# Autodesk Inventor assembly: outer_MIR
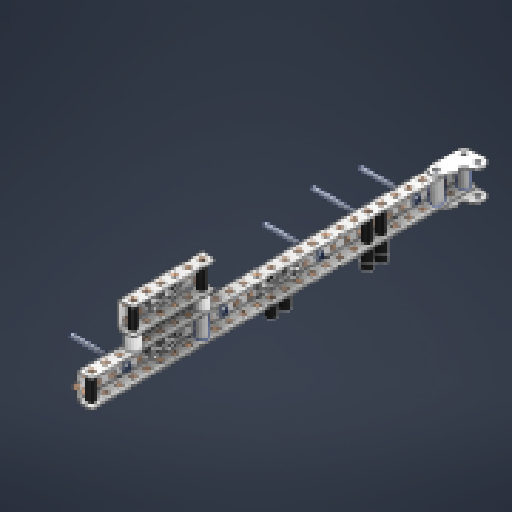
[picture p0: Inventor's stored thumbnail of the model, 512x512]
Saved by Autodesk Inventor 2024 (Build 280153000, 153)
## iProperties
Created: 2023-10-18
Part Number: outer_MIR
Document SubType Name: Assembly
Designer: Averey Ku
Author: avere
## Documents named in this file (16)
- D:\vex_robotics\hardware\cad\goated_v0.1\chassis\mirrored_parts\outer_MIR.iam
- D:\vex_robotics\hardware\cad\goated_v0.1\chassis\mirrored_parts\Alu C 1x2x1x28_MIR.ipt
- D:\vex_robotics\hardware\cad\goated_v0.1\chassis\mirrored_parts\Alu C 1x2x1x6_MIR.ipt
- D:\vex_robotics\hardware\cad\goated_v0.1\chassis\mirrored_parts\lightweight_offset_bearing_MIR.iam
- D:\vex_robotics\hardware\cad\goated_v0.1\chassis\mirrored_parts\.375 OD Aluminum Spacer 0.875_MIR.ipt
- D:\vex_robotics\hardware\cad\VEX-CAD-Inventor-1.41\Structure\Standoff\Standoff .875.ipt
- D:\vex_robotics\hardware\cad\VEX-CAD-Inventor-1.41\Structure\Standoff.ipt
- D:\vex_robotics\hardware\cad\goated_v0.1\chassis\mirrored_parts\lightweight_bearing_MIR.iam
- D:\vex_robotics\hardware\cad\VEX-CAD-Inventor-1.41\Motion\Spacers\Spacer Nylon .375 OD\NSpacer .375 OD x .500.ipt
- D:\vex_robotics\hardware\cad\VEX-CAD-Inventor-1.41\Motion\Spacers\Spacer Nylon .375 OD.ipt
- D:\vex_robotics\hardware\cad\VEX-CAD-Inventor-1.41\Structure\Hardware\Screw Shoulder Robosource\SScrew Shoulder Smooth 2.000 x .04.ipt
- D:\vex_robotics\hardware\cad\VEX-CAD-Inventor-1.41\Structure\Hardware\Screw Shoulder Robosource.ipt
- D:\vex_robotics\hardware\cad\VEX-CAD-Inventor-1.41\Motion\Spacers\Spacer Nylon .500 OD\NSpacer White .500 OD x .500.ipt
- D:\vex_robotics\hardware\cad\VEX-CAD-Inventor-1.41\Motion\Spacers\Spacer Nylon .500 OD.ipt
- D:\vex_robotics\hardware\cad\goated_v0.1\chassis\mirrored_parts\wing_pivot_MIR.ipt
- D:\vex_robotics\hardware\cad\VEX-CAD-Inventor-1.41\Motion\Spacers\Spacer Nylon .375 OD\NSpacer .375 OD x .250.ipt
## Components (28 placed, 11 different names)
1. Alu C 1x2x1x28_MIR:1 — Mate:1, Insert:1, Insert:3, Mate:3, Insert:7, Mate:4, Insert:8, Insert:9, Insert:10, Insert:11, Insert:12, Insert:13, Insert:14, Insert:15, Insert:18, Insert:17, Insert:19, Insert:20, Insert:21, Mate:5, Insert:22, Insert:23, Mate:6, Insert:24, Insert:25, Insert:27, Insert:26
2. Alu C 1x2x1x6_MIR:1 — Mate:1, Insert:1, Mate:2, Insert:2, Insert:5, Insert:6
3. lightweight_offset_bearing_MIR:1 [sub-assembly] — Mate:2, Insert:2
4. .375 OD Aluminum Spacer 0.875_MIR:1 — Insert:3
5. Standoff .875:1 — Insert:5
6. Standoff .875:2 — Insert:6
7. lightweight_offset_bearing_MIR:2 [sub-assembly] — Mate:3, Insert:7
8. lightweight_bearing_MIR:1 [sub-assembly] — Mate:4, Insert:8
9. NSpacer .375 OD x .500:1 — Insert:9, Insert:26
10. NSpacer .375 OD x .500:2 — Insert:10, Insert:27
11. Standoff .875:3 — Insert:11
12. Standoff .875:4 — Insert:12
13. SScrew Shoulder Smooth 2.000 x .04:1 — Insert:13
14. SScrew Shoulder Smooth 2.000 x .04:2 — Insert:14
15. SScrew Shoulder Smooth 2.000 x .04:3 — Insert:15
16. SScrew Shoulder Smooth 2.000 x .04:4 — Insert:18
17. SScrew Shoulder Smooth 2.000 x .04:5 — Insert:17
18. NSpacer White .500 OD x .500:1 — Insert:19
19. NSpacer White .500 OD x .500:2 — Insert:20
20. .375 OD Aluminum Spacer 0.875_MIR:2 — Insert:21
21. wing_pivot_MIR:1 — Mate:5, Insert:22
22. .375 OD Aluminum Spacer 0.875_MIR:3 — Insert:23
23. wing_pivot_MIR:2 — Mate:6, Insert:24
24. Standoff .875:5 — Insert:25
25. NSpacer .375 OD x .500:3 — Insert:27
26. NSpacer .375 OD x .500:4 — Insert:26
27. NSpacer .375 OD x .250:5 — Insert:26
28. NSpacer .375 OD x .250:6 — Insert:27
## Relationships (33: Insert 27, Mate 6)
- Mate:1: Alu C 1x2x1x28_MIR:1 ↔ Alu C 1x2x1x6_MIR:1
- Insert:1 (12.7 mm): Alu C 1x2x1x28_MIR:1 ↔ Alu C 1x2x1x6_MIR:1
- Mate:2: Alu C 1x2x1x6_MIR:1 ↔ lightweight_offset_bearing_MIR:1
- Insert:2: Alu C 1x2x1x6_MIR:1 ↔ lightweight_offset_bearing_MIR:1
- Insert:3: Alu C 1x2x1x28_MIR:1 ↔ .375 OD Aluminum Spacer 0.875_MIR:1
- Insert:5: Alu C 1x2x1x6_MIR:1 ↔ Standoff .875:1
- Insert:6: Alu C 1x2x1x6_MIR:1 ↔ Standoff .875:2
- Mate:3: Alu C 1x2x1x28_MIR:1 ↔ lightweight_offset_bearing_MIR:2
- Insert:7: Alu C 1x2x1x28_MIR:1 ↔ lightweight_offset_bearing_MIR:2
- Mate:4: Alu C 1x2x1x28_MIR:1 ↔ lightweight_bearing_MIR:1
- Insert:8: Alu C 1x2x1x28_MIR:1 ↔ lightweight_bearing_MIR:1
- Insert:9: Alu C 1x2x1x28_MIR:1 ↔ NSpacer .375 OD x .500:1
- Insert:10: Alu C 1x2x1x28_MIR:1 ↔ NSpacer .375 OD x .500:2
- Insert:11: Alu C 1x2x1x28_MIR:1 ↔ Standoff .875:3
- Insert:12: Alu C 1x2x1x28_MIR:1 ↔ Standoff .875:4
- Insert:13: Alu C 1x2x1x28_MIR:1 ↔ SScrew Shoulder Smooth 2.000 x .04:1
- Insert:14: Alu C 1x2x1x28_MIR:1 ↔ SScrew Shoulder Smooth 2.000 x .04:2
- Insert:15: Alu C 1x2x1x28_MIR:1 ↔ SScrew Shoulder Smooth 2.000 x .04:3
- Insert:18: Alu C 1x2x1x28_MIR:1 ↔ SScrew Shoulder Smooth 2.000 x .04:4
- Insert:17: Alu C 1x2x1x28_MIR:1 ↔ SScrew Shoulder Smooth 2.000 x .04:5
- Insert:19: Alu C 1x2x1x28_MIR:1 ↔ NSpacer White .500 OD x .500:1
- Insert:20: Alu C 1x2x1x28_MIR:1 ↔ NSpacer White .500 OD x .500:2
- Insert:21: Alu C 1x2x1x28_MIR:1 ↔ .375 OD Aluminum Spacer 0.875_MIR:2
- Mate:5: Alu C 1x2x1x28_MIR:1 ↔ wing_pivot_MIR:1
- Insert:22: Alu C 1x2x1x28_MIR:1 ↔ wing_pivot_MIR:1
- Insert:23: Alu C 1x2x1x28_MIR:1 ↔ .375 OD Aluminum Spacer 0.875_MIR:3
- Mate:6: Alu C 1x2x1x28_MIR:1 ↔ wing_pivot_MIR:2
- Insert:24: Alu C 1x2x1x28_MIR:1 ↔ wing_pivot_MIR:2
- Insert:25: Alu C 1x2x1x28_MIR:1 ↔ Standoff .875:5
- Insert:27: Alu C 1x2x1x28_MIR:1 ↔ NSpacer .375 OD x .500:3
- Insert:26: Alu C 1x2x1x28_MIR:1 ↔ NSpacer .375 OD x .500:4
- Insert:26: NSpacer .375 OD x .500:1 ↔ NSpacer .375 OD x .250:5
- Insert:27: NSpacer .375 OD x .500:2 ↔ NSpacer .375 OD x .250:6
